# Autodesk Inventor assembly: Arm3
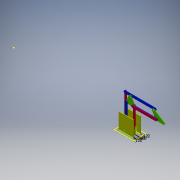
[picture p0: Inventor's stored thumbnail of the model, 180x180]
Saved by Autodesk Inventor 2016 (Build 200138000, 138)
## iProperties
Created: 2017-09-07
Part Number: Arm3
Document SubType Name: Assembly
Designer: student
Author: student
## Documents named in this file (13)
- C:\Users\student\Documents\Inventor Files\arm2\Arm3.iam
- C:\Users\student\Documents\Inventor Files\arm2\part2.ipt
- C:\Users\student\Documents\Inventor Files\arm2\part3.ipt
- C:\Users\student\Documents\Inventor Files\arm2\part4.ipt
- C:\Users\student\Documents\Inventor Files\arm2\part5.ipt
- C:\Users\student\Documents\Inventor Files\arm2\part6.ipt
- C:\Users\student\Documents\Inventor Files\arm2\part7.ipt
- C:\Users\student\Documents\Inventor Files\arm2\part8.ipt
- C:\Users\student\Documents\Inventor Files\arm2\part10.ipt
- C:\Users\student\Documents\Inventor Files\arm2\part11.ipt
- C:\Users\student\Documents\Inventor Files\arm2\arm2_12.ipt
- C:\Users\student\Documents\Inventor Files\arm2\arm2_13.ipt
- C:\Users\student\Documents\Inventor Files\arm2\arm2_14.ipt
## Components (14 placed, 12 different names)
1. part2:1 — Rigid:1, Rotational:6, Rigid:2
2. part3:1 — Rigid:1, Angle:1
3. part4:1 — Rotational:3, Rotational:5, Angle:3, Rotational:6, Rotational:10
4. part5:1 — Rotational:9
5. part6:1 — Rotational:3, Angle:4, Rotational:7, Rotational:9
6. part2:2 — Rotational:5, Angle:2, Rigid:3
7. part3:2 — Rotational:7, Angle:5, Rotational:8
8. part7:1 — Rotational:8, Angle:6, Rigid:4
9. part8:1 — Rotational:10, Angle:7, Rigid:5
10. part10:1 — Rigid:2
11. part11:1 — Rigid:3
12. arm2_12:1 — Rigid:4
13. arm2_13:1 — Rigid:5, Flush:1
14. arm2_14:1 — Flush:1
## Relationships (20: Angle 7, RevoluteJoint 7, WeldJoint 5, Flush 1)
- Rigid:1 [WeldJoint]: part2:1 ↔ part3:1
- Angle:1 (0 deg): part3:1
- Rotational:3 [RevoluteJoint] (-6.35 mm): part4:1 ↔ part6:1
- Rotational:5 [RevoluteJoint]: part4:1 ↔ part2:2
- Angle:2 (180 deg): part2:2
- Angle:3 (0 deg): part4:1
- Angle:4 (180 deg): part6:1
- Rotational:6 [RevoluteJoint]: part2:1 ↔ part4:1
- Rotational:7 [RevoluteJoint]: part6:1 ↔ part3:2
- Angle:5 (180 deg): part3:2
- Rotational:8 [RevoluteJoint]: part3:2 ↔ part7:1
- Angle:6 (0 deg): part7:1
- Rotational:9 [RevoluteJoint] (6.35 mm): part5:1 ↔ part6:1
- Rotational:10 [RevoluteJoint]: part4:1 ↔ part8:1
- Angle:7 (0 deg): part8:1
- Rigid:2 [WeldJoint]: part2:1 ↔ part10:1
- Rigid:3 [WeldJoint] (-6.35 mm): part2:2 ↔ part11:1
- Rigid:4 [WeldJoint] (-6.35 mm): part7:1 ↔ arm2_12:1
- Rigid:5 [WeldJoint]: part8:1 ↔ arm2_13:1
- Flush:1 (3.175 mm): arm2_13:1 ↔ arm2_14:1
